# Autodesk Inventor assembly: splitter_all
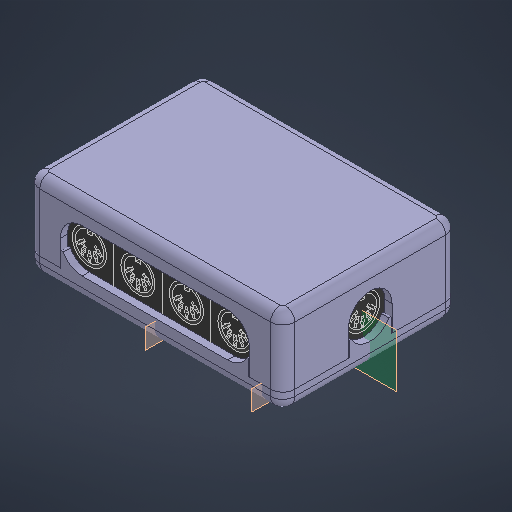
[picture p0: Inventor's stored thumbnail of the model, 512x512]
Saved by Autodesk Inventor 2025.2 (Build 292293000, 293)
## iProperties
Created: 2025-10-04
Part Number: splitter_all
Document SubType Name: Assembly
Designer: micyg
Author: micyg
## Documents named in this file (5)
- D:\Projects\AnotherMidiSplitterV2\Mechanical\splitter_all.iam
- D:\Projects\AnotherMidiSplitterV2\Mechanical\case2.ipt
- D:\Projects\AnotherMidiSplitterV2\Mechanical\mounting.ipt
- D:\Projects\AnotherMidiSplitterV2\Mechanical\Boards\AnotherMidiSplitterV2\AnotherMidiSplitterV2.iam
- D:\Projects\AnotherMidiSplitterV2\Mechanical\case1.ipt
## Components (7 placed, 4 different names)
1. case2:1 — Mate:19, Mate:20, Mate:21, Mate:23, Mate:28, Mate:29, Mate:30, Mate:31, Mate:34
2. mounting:1 — Mate:20, Mate:22, Mate:25, Mate:29
3. mounting:2 — Mate:17, Mate:18, Mate:21, Mate:26, Mate:31
4. mounting:3 — Mate:23, Mate:24, Mate:30
5. mounting:4 — Mate:19, Mate:27, Mate:28
6. AnotherMidiSplitterV2:1 [sub-assembly] — Mate:17, Mate:18, Mate:22, Mate:24, Mate:25, Mate:26, Mate:27, Mate:32, Mate:33
7. case1:1 — Mate:32, Mate:33, Mate:34
## Relationships (18: Mate 18)
- Mate:17: mounting:2 ↔ AnotherMidiSplitterV2:1
- Mate:18: mounting:2 ↔ AnotherMidiSplitterV2:1
- Mate:19: case2:1 ↔ mounting:4
- Mate:20: case2:1 ↔ mounting:1
- Mate:21: case2:1 ↔ mounting:2
- Mate:22: mounting:1 ↔ AnotherMidiSplitterV2:1
- Mate:23: case2:1 ↔ mounting:3
- Mate:24: mounting:3 ↔ AnotherMidiSplitterV2:1
- Mate:25: mounting:1 ↔ AnotherMidiSplitterV2:1
- Mate:26: mounting:2 ↔ AnotherMidiSplitterV2:1
- Mate:27: mounting:4 ↔ AnotherMidiSplitterV2:1
- Mate:28: case2:1 ↔ mounting:4
- Mate:29: case2:1 ↔ mounting:1
- Mate:30: case2:1 ↔ mounting:3
- Mate:31: case2:1 ↔ mounting:2
- Mate:32: AnotherMidiSplitterV2:1 ↔ case1:1
- Mate:33: AnotherMidiSplitterV2:1 ↔ case1:1
- Mate:34: case2:1 ↔ case1:1
